# Autodesk Inventor assembly: Bottom Assembly Exploded
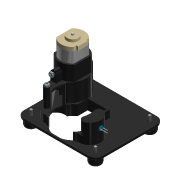
[picture p0: Inventor's stored thumbnail of the model, 180x180]
Saved by Autodesk Inventor 2017 (Build 210142000, 142)
## iProperties
Created: 2016-12-22
Part Number: Bottom Assembly Exploded
Document SubType Name: Assembly
Designer: ge937963
Author: ge937963
## Documents named in this file (9)
- C:\Users\ge937963\Desktop\Inventor View\Bottom Assembly.iam
- C:\Users\ge937963\Desktop\Inventor View\LED.ipt
- C:\Users\ge937963\Desktop\Inventor View\Bottom Plate.ipt
- C:\Users\ge937963\Desktop\Inventor View\Motor Holder.ipt
- C:\Users\ge937963\Desktop\Inventor View\Fan Blade.ipt
- C:\Users\ge937963\Desktop\Inventor View\Screw.ipt
- C:\Users\ge937963\Desktop\Inventor View\Size 130 Motor.ipt
- C:\Users\ge937963\Desktop\Inventor View\Excitation Filter.ipt
- C:\Users\ge937963\Desktop\Inventor View\Spacer.ipt
## Components (17 placed, 8 different names)
1. LED:1 — Mate:1, Tangent:2
2. Bottom Plate:1 — Mate:1, Mate:2, Mate:3, Mate:4, Mate:9, Mate:10, Mate:11, Mate:12, Mate:13, Mate:19, Tangent:2, Mate:22, Mate:23
3. Motor Holder:1 — Mate:2, Mate:3, Mate:5, Mate:6, Mate:7, Mate:8, Angle:1, Mate:18, Mate:19, Mate:20, Mate:21
4. Fan Blade:1 — Mate:4, Mate:18
5. Screw:1 — Mate:5, Flush:1, Mate:20
6. Screw:2 — Mate:6, Flush:1
7. Screw:3 — Mate:7, Tangent:1
8. Size 130 Motor:1 — Mate:8, Angle:1, Mate:21, Tangent:1
9. Excitation Filter:1 — Mate:9, Mate:22
10. Spacer:1 — Mate:10, Flush:2, Flush:3, Mate:15
11. Spacer:2 — Mate:13, Flush:3, Flush:4, Mate:17
12. Spacer:3 — Mate:12, Flush:4, Mate:14, Mate:24
13. Spacer:4 — Mate:11, Flush:2, Mate:16, Mate:23
14. Screw:4 — Flush:5, Mate:16
15. Screw:5 — Flush:5, Flush:6, Mate:15
16. Screw:6 — Flush:6, Flush:7, Mate:17
17. Screw:7 — Flush:7, Mate:14, Mate:24
## Relationships (34: Mate 24, Flush 7, Tangent 2, Angle 1)
- Mate:1: LED:1 ↔ Bottom Plate:1
- Mate:2: Bottom Plate:1 ↔ Motor Holder:1
- Mate:3: Bottom Plate:1 ↔ Motor Holder:1
- Mate:4: Bottom Plate:1 ↔ Fan Blade:1
- Mate:5: Motor Holder:1 ↔ Screw:1
- Mate:6: Motor Holder:1 ↔ Screw:2
- Mate:7: Motor Holder:1 ↔ Screw:3
- Flush:1: Screw:1 ↔ Screw:2
- Mate:8: Motor Holder:1 ↔ Size 130 Motor:1
- Angle:1 (0 deg): Motor Holder:1 ↔ Size 130 Motor:1
- Mate:9: Bottom Plate:1 ↔ Excitation Filter:1
- Mate:10: Bottom Plate:1 ↔ Spacer:1
- Mate:11: Bottom Plate:1 ↔ Spacer:4
- Mate:12: Bottom Plate:1 ↔ Spacer:3
- Mate:13: Bottom Plate:1 ↔ Spacer:2
- Flush:2: Spacer:1 ↔ Spacer:4
- Flush:3: Spacer:1 ↔ Spacer:2
- Flush:4: Spacer:2 ↔ Spacer:3
- Flush:5: Screw:4 ↔ Screw:5
- Flush:6: Screw:5 ↔ Screw:6
- Flush:7: Screw:6 ↔ Screw:7
- Mate:14: Spacer:3 ↔ Screw:7
- Mate:15: Spacer:1 ↔ Screw:5
- Mate:16: Spacer:4 ↔ Screw:4
- Mate:17: Spacer:2 ↔ Screw:6
- Mate:18 (1 mm): Motor Holder:1 ↔ Fan Blade:1
- Mate:19: Bottom Plate:1 ↔ Motor Holder:1
- Mate:20: Motor Holder:1 ↔ Screw:1
- Mate:21: Motor Holder:1 ↔ Size 130 Motor:1
- Tangent:1: Screw:3 ↔ Size 130 Motor:1
- Tangent:2: LED:1 ↔ Bottom Plate:1
- Mate:22: Bottom Plate:1 ↔ Excitation Filter:1
- Mate:23: Bottom Plate:1 ↔ Spacer:4
- Mate:24: Spacer:3 ↔ Screw:7
